# Autodesk Inventor assembly: pitch_motor_flashlight_attached_model
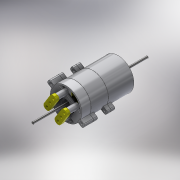
[picture p0: Inventor's stored thumbnail of the model, 180x180]
Saved by Autodesk Inventor 2018 (Build 220112000, 112)
## iProperties
Created: 2018-02-06
Part Number: pitch_motor_flashlight_attached_model
Document SubType Name: Assembly
Designer: mansu
Sending System: SolidWorks 2017
Last Author: leoli
Last Saved: 2018-03-27
Author: mansu
## Documents named in this file (9)
- F:\OneDrive\Documents\2018 UBC\ELEC 391\Controller\cad\release\PitchMotor\pitch_motor_flashlight_attached_model.iam
- F:\OneDrive\Documents\2018 UBC\ELEC 391\Controller\cad\release\PitchMotor\pitch_RotorCore.ipt
- F:\OneDrive\Documents\2018 UBC\ELEC 391\Controller\cad\release\PitchMotor\pitch_shaft.ipt
- F:\OneDrive\Documents\2018 UBC\ELEC 391\Controller\cad\release\PitchMotor\pitch_StatorShell_v5.ipt
- F:\OneDrive\Documents\2018 UBC\ELEC 391\Controller\cad\release\PitchMotor\pitch_StatorShell_v1_Top_Flashlight_attachment.ipt
- F:\OneDrive\Documents\2018 UBC\ELEC 391\Controller\cad\release\PitchMotor\pitch_commutator_attachment1.ipt
- F:\OneDrive\Documents\2018 UBC\ELEC 391\Controller\cad\release\PitchMotor\pitch_stator_front_attachment_flashlight.ipt
- F:\OneDrive\Documents\2018 UBC\ELEC 391\Controller\cad\release\PitchMotor\pitch_pressurecap-front.ipt
- F:\OneDrive\Documents\2018 UBC\ELEC 391\Controller\cad\release\Magnet3010.ipt
## Components (12 placed, 8 different names)
1. pitch_RotorCore:1 — Mate:10, Mate:20
2. pitch_shaft:1 — Mate:9, Mate:10, Mate:11, Mate:12, Mate:15
3. pitch_StatorShell_v5:1 — Mate:1, Mate:2, Flush:1, Mate:3, Mate:4, Flush:2, Mate:5, Mate:6, Flush:3, Mate:7, Mate:8, Flush:4, Mate:9, Mate:16, Mate:19, Mate:20
4. pitch_StatorShell_v1_Top_Flashlight_attachment:1 — Mate:12, Mate:13, Mate:14, Mate:17, Mate:18, Angle:1, Angle:2, Mate:21, Mate:22
5. pitch_commutator_attachment1:1 — Mate:11
6. pitch_stator_front_attachment_flashlight:1 — Mate:15, Mate:16, Mate:17, Mate:18, Mate:19
7. pitch_pressurecap-front:1 — Mate:14, Angle:1, Mate:21
8. pitch_pressurecap-front:2 — Mate:13, Angle:2, Mate:22
9. Magnet3010:1 — Mate:5, Mate:6, Flush:3
10. Magnet3010:2 — Mate:1, Mate:2, Flush:1
11. Magnet3010:3 — Mate:7, Mate:8, Flush:4
12. Magnet3010:4 — Mate:3, Mate:4, Flush:2
## Relationships (28: Mate 22, Flush 4, Angle 2)
- Mate:1: pitch_StatorShell_v5:1 ↔ Magnet3010:2
- Mate:2: pitch_StatorShell_v5:1 ↔ Magnet3010:2
- Flush:1 (2 mm): pitch_StatorShell_v5:1 ↔ Magnet3010:2
- Mate:3: pitch_StatorShell_v5:1 ↔ Magnet3010:4
- Mate:4: pitch_StatorShell_v5:1 ↔ Magnet3010:4
- Flush:2 (2 mm): pitch_StatorShell_v5:1 ↔ Magnet3010:4
- Mate:5: pitch_StatorShell_v5:1 ↔ Magnet3010:1
- Mate:6: pitch_StatorShell_v5:1 ↔ Magnet3010:1
- Flush:3 (2 mm): pitch_StatorShell_v5:1 ↔ Magnet3010:1
- Mate:7: pitch_StatorShell_v5:1 ↔ Magnet3010:3
- Mate:8: pitch_StatorShell_v5:1 ↔ Magnet3010:3
- Flush:4 (2 mm): pitch_StatorShell_v5:1 ↔ Magnet3010:3
- Mate:9: pitch_shaft:1 ↔ pitch_StatorShell_v5:1
- Mate:10: pitch_RotorCore:1 ↔ pitch_shaft:1
- Mate:11: pitch_shaft:1 ↔ pitch_commutator_attachment1:1
- Mate:12: pitch_shaft:1 ↔ pitch_StatorShell_v1_Top_Flashlight_attachment:1
- Mate:13: pitch_StatorShell_v1_Top_Flashlight_attachment:1 ↔ pitch_pressurecap-front:2
- Mate:14: pitch_StatorShell_v1_Top_Flashlight_attachment:1 ↔ pitch_pressurecap-front:1
- Mate:15: pitch_shaft:1 ↔ pitch_stator_front_attachment_flashlight:1
- Mate:16: pitch_StatorShell_v5:1 ↔ pitch_stator_front_attachment_flashlight:1
- Mate:17: pitch_StatorShell_v1_Top_Flashlight_attachment:1 ↔ pitch_stator_front_attachment_flashlight:1
- Mate:18 (0.1 mm): pitch_StatorShell_v1_Top_Flashlight_attachment:1 ↔ pitch_stator_front_attachment_flashlight:1
- Mate:19 (0.1 mm): pitch_StatorShell_v5:1 ↔ pitch_stator_front_attachment_flashlight:1
- Mate:20 (5 mm): pitch_RotorCore:1 ↔ pitch_StatorShell_v5:1
- Angle:1 (0 deg): pitch_StatorShell_v1_Top_Flashlight_attachment:1 ↔ pitch_pressurecap-front:1
- Angle:2 (0 deg): pitch_StatorShell_v1_Top_Flashlight_attachment:1 ↔ pitch_pressurecap-front:2
- Mate:21 (0.1 mm): pitch_StatorShell_v1_Top_Flashlight_attachment:1 ↔ pitch_pressurecap-front:1
- Mate:22 (0.1 mm): pitch_StatorShell_v1_Top_Flashlight_attachment:1 ↔ pitch_pressurecap-front:2
